# Autodesk Inventor assembly: 双四方轴套 头洞
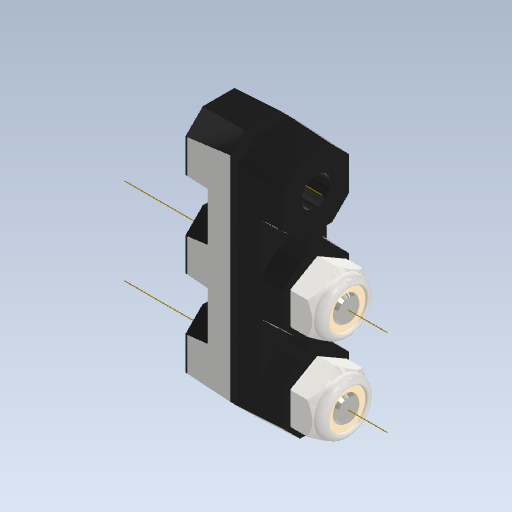
[picture p0: Inventor's stored thumbnail of the model, 512x512]
Saved by Autodesk Inventor 2020 (Build 240168000, 168)
## iProperties
Created: 2019-05-29
Part Number: 双四方轴套 头洞
Document SubType Name: Assembly
Designer: aresp
Mass: 31.199 g
Surface Area: 44.065 cm^2
Volume: 3.98528 cm^3
Density: 7.82856 g/cm^3
Author: aresp
## Documents named in this file (4)
- D:\vault\ncrCadLib\轴相关\细轴配套\双四方轴套 头洞.iam
- D:\vault\ncrCadLib\轴相关\细轴配套\零件\细轴四方轴承.ipt
- D:\vault\ncrCadLib\螺丝螺帽\Screw 8-32 x 0.750'' 五号.ipt
- D:\vault\ncrCadLib\螺丝螺帽\防滑螺帽.ipt
## Components (6 placed, 3 different names)
1. 细轴四方轴承:1 — 配合:1, 配合:2, 配合:3, 配合:6
2. 细轴四方轴承:2 — 配合:1, 配合:2, 配合:3, 配合:7, 配合:9
3. 防滑螺帽:1 — 配合:8, 配合:9
4. Screw 8-32 x 0.750'' 五号:1 — 配合:6, 配合:7, 配合:8
5. 防滑螺帽:2
6. Screw 8-32 x 0.750'' 五号:2
## Component patterns: (2 elements, first: 防滑螺帽:1 + Screw 8-32 x 0.750'' 五号:1)
## Relationships (7: Mate 7)
- 配合:1 [Mate]: 细轴四方轴承:1 ↔ 细轴四方轴承:2
- 配合:2 [Mate]: 细轴四方轴承:1 ↔ 细轴四方轴承:2
- 配合:3 [Mate] (1.5748 mm): 细轴四方轴承:1 ↔ 细轴四方轴承:2
- 配合:6 [Mate]: 细轴四方轴承:1 ↔ Screw 8-32 x 0.750'' 五号:1
- 配合:7 [Mate]: 细轴四方轴承:2 ↔ Screw 8-32 x 0.750'' 五号:1
- 配合:8 [Mate]: 防滑螺帽:1 ↔ Screw 8-32 x 0.750'' 五号:1
- 配合:9 [Mate]: 细轴四方轴承:2 ↔ 防滑螺帽:1
